# Autodesk Inventor assembly: MG-Waveshare Kamera 25x24
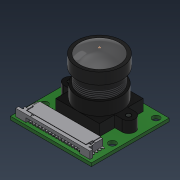
[picture p0: Inventor's stored thumbnail of the model, 180x180]
Saved by Autodesk Inventor 2022.1 (Build 261234020, 234B)
## iProperties
Part Number: MG-Waveshare Kamera 25x24
Material: Generisch
Document SubType Name: Assembly
Designer: rYan
Mass: 2.24165 g
Surface Area: 38.2639 cm^2
Volume: 2.9629 cm^3
Density: 0.756574 g/cm^3
Author: rYan
## Documents named in this file (6)
- D:\TIGERsGIT\Hardware\mechanik\2020\Inventor\Purchased Parts\Waveshare Kamera 25x24\MG-Waveshare Kamera 25x24.iam
- D:\TIGERsGIT\Hardware\mechanik\2020\Inventor\Purchased Parts\Waveshare Kamera 25x24\Waveshare Kamera PCB 24x25.ipt
- D:\TIGERsGIT\Hardware\mechanik\2020\Inventor\Inhaltscenter\de-DE\ISO 7049 - F-Z(1)\DIN EN ISO 7049 - ST2,2 x 4,5 - F - Z.ipt
- D:\TIGERsGIT\Hardware\mechanik\2020\Inventor\Purchased Parts\Waveshare Kamera 25x24\Linse 12mm Typ G.ipt
- D:\TIGERsGIT\Hardware\mechanik\2020\Inventor\Purchased Parts\Waveshare Kamera 25x24\Linsenhalter M12.ipt
- D:\TIGERsGIT\Hardware\mechanik\2020\Inventor\Purchased Parts\Waveshare Kamera 25x24\FPC Conn 15pin 1mm.ipt
## Components (6 placed, 5 different names)
1. Waveshare Kamera PCB 24x25:1 — Einfügen:1, Passend:1, Einfügen:2, Einfügen:3, Fluchtend:1, Fluchtend:2, Fluchtend:3, Passend:4, Fluchtend:4, Fluchtend:5
2. DIN EN ISO 7049 - F-Z ST2,2 x 4,5 - F - Z:2 — Einfügen:2
3. DIN EN ISO 7049 - F-Z ST2,2 x 4,5 - F - Z:3 — Einfügen:3
4. Linse 12mm Typ G:1 — Passend:2, Passend:3
5. Linsenhalter M12:1 — Einfügen:1, Passend:1, Passend:2, Passend:3
6. FPC Conn 15pin 1mm:1 — Passend:4, Fluchtend:4, Fluchtend:5
## Relationships (12: Flush 5, Mate 4, Insert 3)
- Einfügen:1 [Insert]: Waveshare Kamera PCB 24x25:1 ↔ Linsenhalter M12:1
- Passend:1 [Mate]: Waveshare Kamera PCB 24x25:1 ↔ Linsenhalter M12:1
- Einfügen:2 [Insert]: Waveshare Kamera PCB 24x25:1 ↔ DIN EN ISO 7049 - F-Z ST2,2 x 4,5 - F - Z:2
- Einfügen:3 [Insert]: Waveshare Kamera PCB 24x25:1 ↔ DIN EN ISO 7049 - F-Z ST2,2 x 4,5 - F - Z:3
- Fluchtend:1 [Flush]: Waveshare Kamera PCB 24x25:1
- Fluchtend:2 [Flush]: Waveshare Kamera PCB 24x25:1
- Fluchtend:3 [Flush]: Waveshare Kamera PCB 24x25:1
- Passend:2 [Mate]: Linse 12mm Typ G:1 ↔ Linsenhalter M12:1
- Passend:3 [Mate] (4.5 mm): Linse 12mm Typ G:1 ↔ Linsenhalter M12:1
- Passend:4 [Mate]: Waveshare Kamera PCB 24x25:1 ↔ FPC Conn 15pin 1mm:1
- Fluchtend:4 [Flush]: Waveshare Kamera PCB 24x25:1 ↔ FPC Conn 15pin 1mm:1
- Fluchtend:5 [Flush] (0.6 mm): Waveshare Kamera PCB 24x25:1 ↔ FPC Conn 15pin 1mm:1
